# Autodesk Inventor assembly: H54P-200_M54P-060
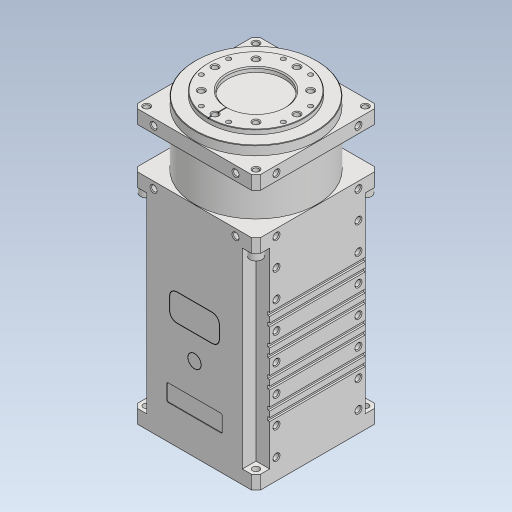
[picture p0: Inventor's stored thumbnail of the model, 512x512]
Saved by Autodesk Inventor 2023 (Build 270158000, 158)
## iProperties
Created: 2023-04-15
Part Number: H54P-200_M54P-060
Document SubType Name: Assembly
Designer: michi
Author: michi
## Documents named in this file (3)
- C:\Users\michi\OneDrive - Kyoto University\lab\6_SHINOBI\FUHGA4\Design_Mechanism\Dynamixel\PH54-200\H54P-200_M54P-060.iam
- C:\Users\michi\OneDrive - Kyoto University\lab\6_SHINOBI\FUHGA4\Design_Mechanism\Dynamixel\PH54-200\H54P-200_M54P-060_body.ipt
- C:\Users\michi\OneDrive - Kyoto University\lab\6_SHINOBI\FUHGA4\Design_Mechanism\Dynamixel\PH54-200\H54P-200_M54P-060_hone.ipt
## Components (2 placed, 2 different names)
1. H54P-200_M54P-060_body:1 — 挿入:1
2. H54P-200_M54P-060_hone:1 — 挿入:1
## Relationships (1: Insert 1)
- 挿入:1 [Insert]: H54P-200_M54P-060_body:1 ↔ H54P-200_M54P-060_hone:1
